# Autodesk Inventor assembly: Assembly2
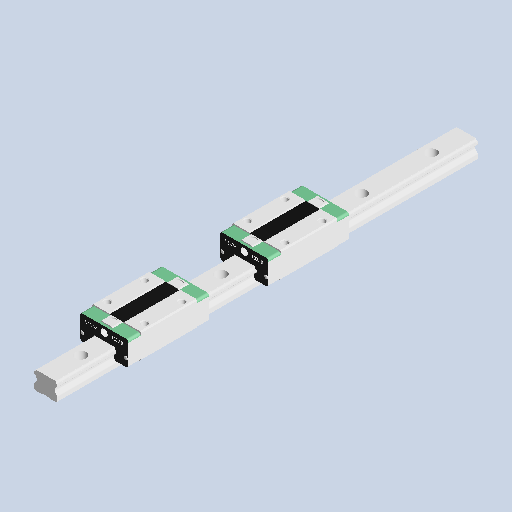
[picture p0: Inventor's stored thumbnail of the model, 512x512]
Saved by Autodesk Inventor 2023 (Build 270158000, 158)
## iProperties
Created: 2025-04-08
Part Number: Assembly2
Document SubType Name: Assembly
Designer: LENOVO
Author: LENOVO
## Documents named in this file (3)
- E:\TAI LIEU\Final_Project\DONE\CoCauTrucZ\Ray_Truot.iam
- E:\TAI LIEU\Final_Project\DONE\CoCauTrucZ\egh20ca_02.ipt
- E:\TAI LIEU\Final_Project\DONE\CoCauTrucZ\egh20ca_01.ipt
## Components (3 placed, 2 different names)
1. egh20ca_02:1 — Mate:1, Mate:2, Mate:3, Mate:4, Flush:1
2. egh20ca_01:1 — Mate:1, Mate:2, Flush:1, Mate:5
3. egh20ca_01:2 — Mate:3, Mate:4, Mate:5
## Relationships (6: Mate 5, Flush 1)
- Mate:1 (-0.07 mm): egh20ca_02:1 ↔ egh20ca_01:1
- Mate:2 (-0.07 mm): egh20ca_02:1 ↔ egh20ca_01:1
- Mate:3 (-0.07 mm): egh20ca_02:1 ↔ egh20ca_01:2
- Mate:4 (-0.07 mm): egh20ca_02:1 ↔ egh20ca_01:2
- Flush:1 (50 mm): egh20ca_02:1 ↔ egh20ca_01:1
- Mate:5 (88 mm): egh20ca_01:1 ↔ egh20ca_01:2
